# Autodesk Inventor assembly: 3A.04.03.JS.74.75mm
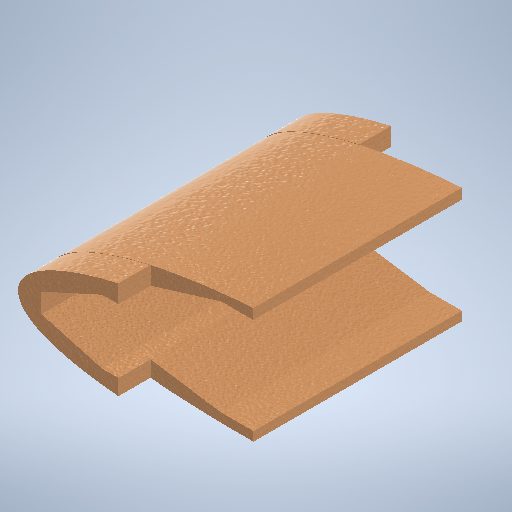
[picture p0: Inventor's stored thumbnail of the model, 512x512]
Saved by Autodesk Inventor 2025.1 (Build 291241000, 241)
## iProperties
Created: 2025-01-14
Part Number: 3A.04.03.JS.74.75mm
Document SubType Name: Assembly
Designer: johan
Author: johan
## Documents named in this file (3)
- C:\Users\johan\OneDrive - University of Bristol\CAD docs\2) Wing\3) Leading edge\assemblies\3A.04.03.JS.74.75mm.iam
- C:\Users\johan\OneDrive - University of Bristol\CAD docs\2) Wing\3) Leading edge\parts\3P.04.03.JS. leading edge 74.75mm.ipt
- C:\Users\johan\OneDrive - University of Bristol\CAD docs\2) Wing\3) Leading edge\parts\3P.04.JS.2414 rib leading edge v2.ipt
## Components (3 placed, 2 different names)
1. 3P.04.03.JS. leading edge 74.75mm:1 — Rigid:1, Rigid:2
2. 3P.04.JS.2414 rib leading edge v2:1 — Rigid:2
3. 3P.04.JS.2414 rib leading edge v2:2 — Rigid:1
## Relationships (2: WeldJoint 2)
- Rigid:1 [WeldJoint]: 3P.04.03.JS. leading edge 74.75mm:1 ↔ 3P.04.JS.2414 rib leading edge v2:2
- Rigid:2 [WeldJoint]: 3P.04.03.JS. leading edge 74.75mm:1 ↔ 3P.04.JS.2414 rib leading edge v2:1
